# Autodesk Inventor assembly: RotorShaft
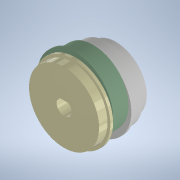
[picture p0: Inventor's stored thumbnail of the model, 180x180]
Saved by Autodesk Inventor 2021 (Build 250183000, 183)
## iProperties
Created: 2022-08-31
Part Number: RotorShaft
Document SubType Name: Assembly
Designer: MicnedSQ
Author: MicnedSQ
## Documents named in this file (4)
- C:\Users\MicnedSQ\Desktop\V1\Base\RotorShaft.iam
- C:\Users\MicnedSQ\Desktop\V1\Base\RotorShaft1.ipt
- C:\Users\MicnedSQ\Desktop\V1\Base\RotorShaft2.ipt
- C:\Users\MicnedSQ\Desktop\V1\Base\RotorShaft3.ipt
## Components (3 placed, 3 different names)
1. RotorShaft1:1 — Sztywne:1
2. RotorShaft2:1 — Sztywne:1, Sztywne:2
3. RotorShaft3:1 — Sztywne:2
## Relationships (2: WeldJoint 2)
- Sztywne:1 [WeldJoint]: RotorShaft1:1 ↔ RotorShaft2:1
- Sztywne:2 [WeldJoint]: RotorShaft2:1 ↔ RotorShaft3:1
